# Autodesk Inventor assembly: HexaBot
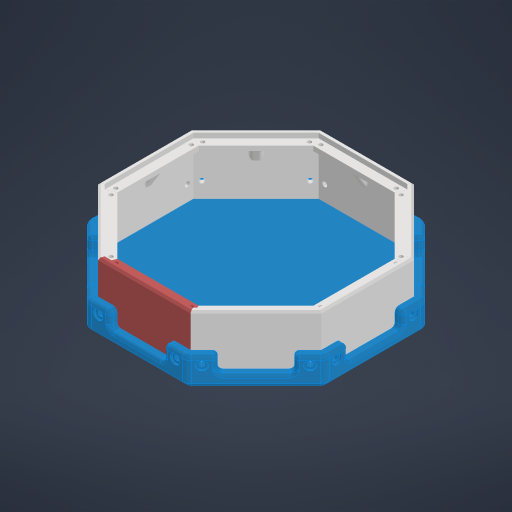
[picture p0: Inventor's stored thumbnail of the model, 512x512]
Saved by Autodesk Inventor 2024.2 (Build 282272000, 272)
## iProperties
Created: 2024-08-28
Part Number: HexaBot
Document SubType Name: Assembly
Designer: SEON06
Author: SEON06
## Documents named in this file (3)
- C:\Users\SEON06\Documents\Inventor\HexaBot_s\HexaBot.iam
- C:\Users\SEON06\Documents\Inventor\HexaBot_s\Base.ipt
- C:\Users\SEON06\Documents\Inventor\HexaBot_s\Wall.ipt
## Components (9 placed, 2 different names)
1. Base:1 — 메이트:1, 각도:1, 메이트:2, 메이트:3, 메이트:5, 메이트:6, 메이트:7, 메이트:8, 메이트:9, 메이트:10, 메이트:11, 메이트:12, 메이트:13, 메이트:14, 메이트:15, 메이트:16, 메이트:17, 메이트:18, 메이트:19, 메이트:20, 메이트:21
2. Wall:1 — 메이트:2, 메이트:3, 메이트:7
3. Wall:2 — 메이트:5, 메이트:6, 메이트:8
4. Wall:3 — 메이트:9, 메이트:10, 메이트:11
5. Wall:4 — 메이트:12, 메이트:17
6. Wall:5 — 메이트:13, 메이트:18
7. Wall:6 — 메이트:15, 메이트:20
8. Wall:7 — 메이트:16, 메이트:19
9. Wall:8 — 메이트:14, 메이트:21
## Relationships (21: Mate 20, Angle 1)
- 메이트:1 [Mate]: Base:1
- 각도:1 [Angle] (0 deg): Base:1
- 메이트:2 [Mate]: Base:1 ↔ Wall:1
- 메이트:3 [Mate]: Base:1 ↔ Wall:1
- 메이트:5 [Mate]: Base:1 ↔ Wall:2
- 메이트:6 [Mate]: Base:1 ↔ Wall:2
- 메이트:7 [Mate]: Base:1 ↔ Wall:1
- 메이트:8 [Mate]: Base:1 ↔ Wall:2
- 메이트:9 [Mate]: Base:1 ↔ Wall:3
- 메이트:10 [Mate]: Base:1 ↔ Wall:3
- 메이트:11 [Mate]: Base:1 ↔ Wall:3
- 메이트:12 [Mate]: Base:1 ↔ Wall:4
- 메이트:13 [Mate]: Base:1 ↔ Wall:5
- 메이트:14 [Mate]: Base:1 ↔ Wall:8
- 메이트:15 [Mate]: Base:1 ↔ Wall:6
- 메이트:16 [Mate]: Base:1 ↔ Wall:7
- 메이트:17 [Mate]: Base:1 ↔ Wall:4
- 메이트:18 [Mate]: Base:1 ↔ Wall:5
- 메이트:19 [Mate]: Base:1 ↔ Wall:7
- 메이트:20 [Mate]: Base:1 ↔ Wall:6
- 메이트:21 [Mate]: Base:1 ↔ Wall:8
